# Autodesk Inventor assembly: WaterBlock
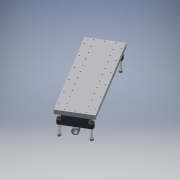
[picture p0: Inventor's stored thumbnail of the model, 180x180]
Saved by Autodesk Inventor 2019.4 (Build 234330000, 330)
## iProperties
Created: 2020-04-27
Part Number: WaterBlock
Document SubType Name: Assembly
Designer: Ed
Author: Ed
## Documents named in this file (7)
- C:\Users\Ed\Dropbox\Ed's Omax\deBivort\heat gradient\Inventor\WaterBlock.iam
- C:\Users\Ed\Dropbox\Ed's Omax\deBivort\heat gradient\Inventor\PVCBottom.ipt
- C:\Users\Ed\Dropbox\Ed's Omax\deBivort\heat gradient\Inventor\Gasket.ipt
- C:\Users\Ed\Dropbox\Ed's Omax\deBivort\heat gradient\Inventor\PVCmiddle.ipt
- C:\Users\Ed\Dropbox\Ed's Omax\deBivort\heat gradient\Inventor\AlTop.ipt
- C:\Users\Ed\Dropbox\Ed's Omax\deBivort\heat gradient\Inventor\TubeFitting.ipt
- C:\Users\Ed\Dropbox\Ed's Omax\deBivort\heat gradient\Inventor\1420feet.ipt
## Components (11 placed, 6 different names)
1. PVCBottom:1 — Mate:1, Mate:2, Mate:3, Mate:13, Mate:14, Mate:15, Mate:16, Mate:18, Mate:20, Flush:18, Mate:21
2. Gasket:1 — Mate:1, Mate:2, Mate:3, Mate:4, Mate:5, Mate:6
3. PVCmiddle:1 — Mate:4, Mate:5, Mate:6, Mate:7, Mate:8, Mate:9
4. Gasket:2 — Mate:7, Mate:8, Mate:9, Mate:10, Mate:11, Mate:12
5. AlTop:1 — Mate:10, Mate:11, Mate:12
6. TubeFitting:1 — Mate:13, Flush:22, Mate:21
7. TubeFitting:2 — Mate:14, Flush:22
8. 1420feet:1 — Mate:20, Flush:18, Flush:19, Flush:20, Flush:21
9. 1420feet:2 — Mate:18, Flush:19
10. 1420feet:3 — Mate:16, Flush:20
11. 1420feet:4 — Mate:15, Flush:21
## Relationships (24: Mate 19, Flush 5)
- Mate:1: PVCBottom:1 ↔ Gasket:1
- Mate:2: PVCBottom:1 ↔ Gasket:1
- Mate:3: PVCBottom:1 ↔ Gasket:1
- Mate:4: Gasket:1 ↔ PVCmiddle:1
- Mate:5: Gasket:1 ↔ PVCmiddle:1
- Mate:6: Gasket:1 ↔ PVCmiddle:1
- Mate:7: PVCmiddle:1 ↔ Gasket:2
- Mate:8: PVCmiddle:1 ↔ Gasket:2
- Mate:9: PVCmiddle:1 ↔ Gasket:2
- Mate:10: Gasket:2 ↔ AlTop:1
- Mate:11: Gasket:2 ↔ AlTop:1
- Mate:12: Gasket:2 ↔ AlTop:1
- Mate:13: PVCBottom:1 ↔ TubeFitting:1
- Mate:14: PVCBottom:1 ↔ TubeFitting:2
- Mate:15: PVCBottom:1 ↔ 1420feet:4
- Mate:16: PVCBottom:1 ↔ 1420feet:3
- Mate:18: PVCBottom:1 ↔ 1420feet:2
- Mate:20: PVCBottom:1 ↔ 1420feet:1
- Flush:18 (38.1 mm): PVCBottom:1 ↔ 1420feet:1
- Flush:19: 1420feet:1 ↔ 1420feet:2
- Flush:20: 1420feet:1 ↔ 1420feet:3
- Flush:21: 1420feet:1 ↔ 1420feet:4
- Flush:22: TubeFitting:1 ↔ TubeFitting:2
- Mate:21: PVCBottom:1 ↔ TubeFitting:1
